# Autodesk Inventor assembly: nc_nhk1
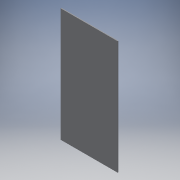
[picture p0: Inventor's stored thumbnail of the model, 180x180]
Saved by Autodesk Inventor 2019 (Build 230136000, 136)
## iProperties
Created: 2022-02-19
Part Number: nc_nhk1
Material: 一般
Document SubType Name: Assembly
Designer: yuta
Author: yuta
## Documents named in this file (3)
- C:\Users\yuta\Documents\キャチロボ\nc_nhk1.iam
- C:\Users\yuta\Documents\キャチロボ\NC.port.ipt
- C:\Users\yuta\Documents\キャチロボ\nhk24.ipt
## Components (5 placed, 2 different names)
1. NC.port:1 — メイト:1, フラッシュ:1, フラッシュ:2, メイト:2, メイト:3, メイト:4, フラッシュ:3, フラッシュ:4, フラッシュ:5
2. nhk24:1 — メイト:1, フラッシュ:1, フラッシュ:2, メイト:5
3. nhk24:2 — メイト:2, フラッシュ:3, メイト:5, メイト:6
4. nhk24:3 — メイト:3, フラッシュ:4, メイト:6, メイト:7
5. nhk24:4 — メイト:4, フラッシュ:5, メイト:7
## Relationships (12: Mate 7, Flush 5)
- メイト:1 [Mate]: NC.port:1 ↔ nhk24:1
- フラッシュ:1 [Flush] (5 mm): NC.port:1 ↔ nhk24:1
- フラッシュ:2 [Flush] (5 mm): NC.port:1 ↔ nhk24:1
- メイト:2 [Mate]: NC.port:1 ↔ nhk24:2
- メイト:3 [Mate]: NC.port:1 ↔ nhk24:3
- メイト:4 [Mate]: NC.port:1 ↔ nhk24:4
- フラッシュ:3 [Flush] (5 mm): NC.port:1 ↔ nhk24:2
- メイト:5 [Mate] (8 mm): nhk24:1 ↔ nhk24:2
- フラッシュ:4 [Flush] (5 mm): NC.port:1 ↔ nhk24:3
- メイト:6 [Mate] (8 mm): nhk24:2 ↔ nhk24:3
- フラッシュ:5 [Flush] (5 mm): NC.port:1 ↔ nhk24:4
- メイト:7 [Mate] (8 mm): nhk24:3 ↔ nhk24:4
